# Autodesk Inventor assembly: robotArmWithWormGearBoxAndSprockets
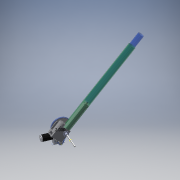
[picture p0: Inventor's stored thumbnail of the model, 180x180]
Saved by Autodesk Inventor 2018.2 (Build 222227000, 227)
## iProperties
Created: 2017-04-29
Part Number: robotArmWithWormGearBoxAndSprockets
Document SubType Name: Assembly
Designer: steele
Author: steele
## Documents named in this file (7)
- D:\snobotics\CAD-Development\robSteele\2018-FRC\GripperArm\robotArmWithWormGearBoxAndSprockets.iam
- D:\snobotics\CAD-Development\robSteele\SnoBotics2017\Arm\am-0917+WormBox.iam
- D:\snobotics\CAD-Development\robSteele\SnoBotics2017\Arm\am-2099+Collar+Clamp,+0.5''+Bore,+Aluminum.iam
- D:\snobotics\CAD-Development\robSteele\SnoBotics2017\Arm\robotArmWithWormGearBox\Design Accelerator\Bolted Connection1.iam
- D:\snobotics\CAD-Development\robSteele\2018-FRC\GripperArm\robotArmWithWormGearBoxAndSprockets\Design Accelerator\Chain Drive1.iam
- D:\snobotics\CAD-Development\robSteele\2018-FRC\GripperArm\1_2_inchShaftForArm.ipt
- D:\snobotics\CAD-Development\robSteele\2018-FRC\GripperArm\linearActuatorWithPvcArm.iam
## Components (7 placed, 6 different names)
1. am-0917+WormBox:1 [sub-assembly] — Flush:1
2. am-2099+Collar+Clamp,+0.5''+Bore,+Aluminum:1 [sub-assembly]
3. Bolted Connection:1 [sub-assembly]
4. Chain Drive:1 [sub-assembly] — Mate:1, Mate:2, Insert:1
5. 1_2_inchShaftForArm:1 — Mate:1, Mate:2
6. linearActuatorWithPvcArm:1 [sub-assembly] — Insert:1, Insert:2
7. 1_2_inchShaftForArm:2 — Insert:2
## Relationships (5: Mate 2, Insert 2, Flush 1)
- Flush:1 (12.7 mm): am-0917+WormBox:1
- Mate:1: Chain Drive:1 ↔ 1_2_inchShaftForArm:1
- Mate:2: Chain Drive:1 ↔ 1_2_inchShaftForArm:1
- Insert:1 (-25.4 mm): Chain Drive:1 ↔ linearActuatorWithPvcArm:1
- Insert:2: linearActuatorWithPvcArm:1 ↔ 1_2_inchShaftForArm:2
